# Autodesk Inventor assembly: thumbL1
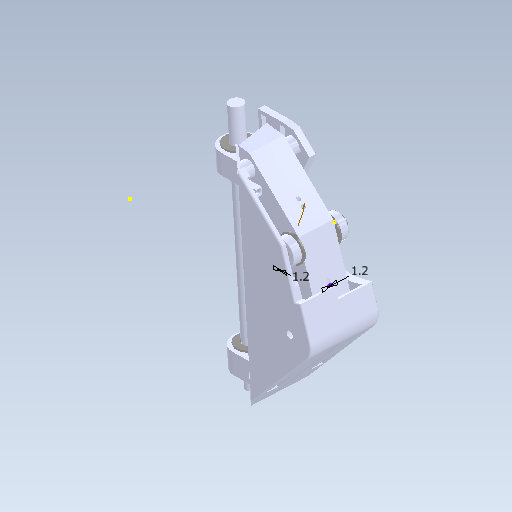
[picture p0: Inventor's stored thumbnail of the model, 512x512]
Saved by Autodesk Inventor 2020 (Build 240168000, 168)
## iProperties
Created: 2020-04-30
Part Number: thumbL1
Document SubType Name: Assembly
Designer: sami_
Author: sami_
## Documents named in this file (9)
- C:\Users\sami_\Documents\V1.6\thumbL1.iam
- C:\Users\sami_\Documents\V1.6\Workgroups\NotInProject\Palm\Part3.ipt
- C:\Users\sami_\Documents\V1.6\Workgroups\NotInProject\Palm\Front Cover.ipt
- C:\Users\sami_\Documents\V1.6\Workgroups\NotInProject\Palm\Back Cover.ipt
- C:\Users\sami_\Documents\V1.6\Workgroups\NotInProject\Palm\Bearing4mm Basic.ipt
- C:\Users\sami_\Documents\V1.6\Workgroups\NotInProject\ISO 7092 - ST 4 - 140 HV.ipt
- C:\Users\sami_\Documents\V1.6\Libraries\Content Center Files\en-US\ISO 1224-1 M\ISO 1224-1 - 17 - 4 x 7 x 2.ipt
- C:\Users\sami_\Documents\V1.6\Workgroups\NotInProject\Palm\Part2-2.ipt
- C:\Users\sami_\Documents\V1.6\Workgroups\NotInProject\Palm\SHAFT2.ipt
## Components (14 placed, 8 different names)
1. Part3:1
2. Front Cover:1
3. Back Cover:1
4. Bearing4mm Basic:1
5. Bearing4mm Basic:2
6. ISO 7092 ST 4 - 140 HV:1
7. ISO 7092 ST 4 - 140 HV:2
8. ISO 1224-1 (Metric) 17 - 4 x 7 x 2:1
9. ISO 7092 ST 4 - 140 HV:3
10. ISO 7092 ST 4 - 140 HV:4
11. ISO 7092 ST 4 - 140 HV:5
12. ISO 7092 ST 4 - 140 HV:6
13. Part2-2:1
14. SHAFT2:1
## Relationships (17: Mate 14, WeldJoint 3)
- [WeldJoint]: Bearing4mm Basic:1 ↔ ISO 7092 ST 4 - 140 HV:2
- [WeldJoint]: Bearing4mm Basic:2 ↔ ISO 7092 ST 4 - 140 HV:1
- [Mate]: Front Cover:1 ↔ Part2-2:1
- [Mate]: Front Cover:1 ↔ Part2-2:1
- [Mate]: Front Cover:1 ↔ Part2-2:1
- [Mate]: Back Cover:1 ↔ Part2-2:1
- [Mate]: Back Cover:1 ↔ Part2-2:1
- [Mate]: Back Cover:1 ↔ Part2-2:1
- [Mate]: ISO 1224-1 (Metric) 17 - 4 x 7 x 2:1 ↔ Part2-2:1
- [WeldJoint]: ISO 1224-1 (Metric) 17 - 4 x 7 x 2:1 ↔ Part2-2:1
- [Mate]: Bearing4mm Basic:2 ↔ SHAFT2:1
- [Mate] (-1.175 mm): Bearing4mm Basic:2 ↔ SHAFT2:1
- [Mate]: ISO 7092 ST 4 - 140 HV:3 ↔ Part2-2:1
- [Mate]: Part2-2:1 ↔ SHAFT2:1
- [Mate]: ISO 7092 ST 4 - 140 HV:1 ↔ Part2-2:1
- [Mate]: Bearing4mm Basic:1 ↔ SHAFT2:1
- [Mate]: ISO 7092 ST 4 - 140 HV:2 ↔ Part2-2:1
